# Autodesk Inventor assembly: Assembly_Cube_empty_withBase
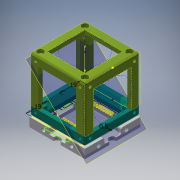
[picture p0: Inventor's stored thumbnail of the model, 180x180]
Saved by Autodesk Inventor 2019 (Build 230136000, 136)
## iProperties
Created: 2019-08-09
Part Number: Assembly_Cube_empty_withBase
Document SubType Name: Assembly
Designer: marsikovabarbora
Author: marsikovabarbora
## Documents named in this file (3)
- D:\Dropbox\UC2\02_CAD\INVENTOR\uc2_v2\Assembly_Cube_empty_withBase.iam
- D:\Dropbox\UC2\02_CAD\INVENTOR\uc2_v2\Assembly_Cube_empty_1x1_v2.iam
- D:\Dropbox\UC2\02_CAD\INVENTOR\uc2_v2\Assembly_Base_1x1_Magnets.iam
## Components (2 placed, 2 different names)
1. Assembly_Cube_empty_1x1_v2:1 [sub-assembly] — Mate:3, Angle:1, Mate:4
2. Assembly_Base_1x1_Magnets:1 [sub-assembly] — Mate:1, Mate:2, Mate:3, Angle:1, Mate:4, Angle:2
## Relationships (6: Mate 4, Angle 2)
- Mate:1: Assembly_Base_1x1_Magnets:1
- Mate:2: Assembly_Base_1x1_Magnets:1
- Mate:3: Assembly_Cube_empty_1x1_v2:1 ↔ Assembly_Base_1x1_Magnets:1
- Angle:1 (0 deg): Assembly_Cube_empty_1x1_v2:1 ↔ Assembly_Base_1x1_Magnets:1
- Mate:4 (1 mm): Assembly_Cube_empty_1x1_v2:1 ↔ Assembly_Base_1x1_Magnets:1
- Angle:2 (0 deg): Assembly_Base_1x1_Magnets:1
